# Autodesk Inventor assembly: Chain Drive
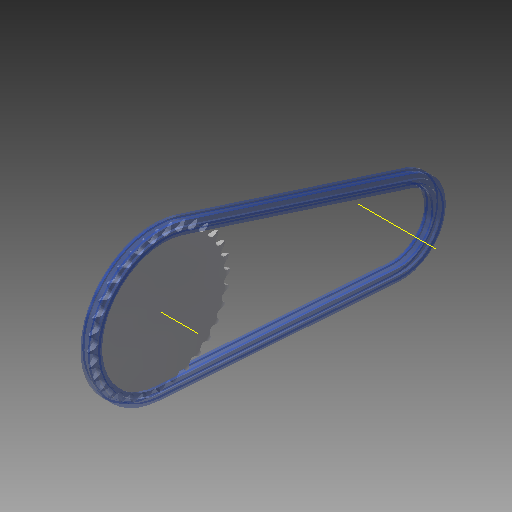
[picture p0: Inventor's stored thumbnail of the model, 512x512]
Saved by Autodesk Inventor 2019.4 (Build 234330000, 330)
## iProperties
Created: 2019-12-07
Part Number: Chain Drive
Document SubType Name: Assembly
Designer: admin
ClientObjectVersion: 1
Author: admin
## Documents named in this file (3)
- C:\Users\admin\Desktop\FRC 2020 Engineering\GitHub\7738-CAD-prep\WCD\WCD V2\Design Accelerator\Chain Drive2.iam
- C:\Users\admin\Desktop\FRC 2020 Engineering\GitHub\7738-CAD-prep\WCD\WCD V2\Design Accelerator\Roller Chain2.ipt
- C:\Users\admin\Desktop\FRC 2020 Engineering\GitHub\7738-CAD-prep\WCD\WCD V2\Design Accelerator\Roller Chain Sprocket22.ipt
## Components (2 placed, 2 different names)
1. Roller Chain:1 — Flush:1, Mate:1, Mate:2
2. Roller Chain Sprocket2:1 — Flush:1, Mate:1, Mate:2
## Relationships (3: Mate 2, Flush 1)
- Flush:1: Roller Chain:1 ↔ Roller Chain Sprocket2:1
- Mate:1: Roller Chain:1 ↔ Roller Chain Sprocket2:1
- Mate:2: Roller Chain:1 ↔ Roller Chain Sprocket2:1
